# Autodesk Inventor assembly: Zlozenie_smc
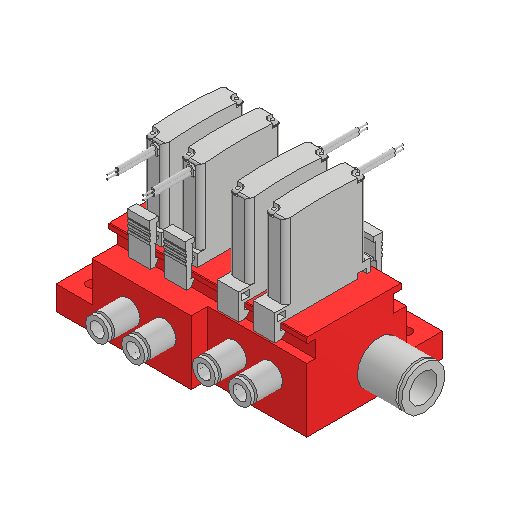
[picture p0: Inventor's stored thumbnail of the model, 512x512]
Saved by Autodesk Inventor 2024.3 (Build 283343000, 343)
## iProperties
Created: 2025-06-09
Part Number: Zlozenie_smc
Document SubType Name: Assembly
Designer: MPA
Author: MPA
## Documents named in this file (5)
- C:\MPA - shortPath\magisterka\V3\Workspace\Zlozenie_smc.iam
- C:\MPA - shortPath\magisterka\V3\Workspace\Zakupowe\smc\SX12F-KH.ipt
- C:\MPA - shortPath\magisterka\V3\Workspace\Plyta_SMC.ipt
- C:\MPA - shortPath\magisterka\V3\Workspace\Zakupowe\smc\KQ2S06-01AS_(A) Brass.ipt
- C:\MPA - shortPath\magisterka\V3\Workspace\Zakupowe\smc\KQ2S12-02AS_(A) Brass.ipt
## Components (10 placed, 4 different names)
1. Plyta_SMC:1 — Flush:1, Flush:2, Flush:3, Insert:1, Mate:1, Insert:2, Mate:2, Insert:3, Insert:4, Insert:5
2. KQ2S12-02AS_(A) Brass:1 — Insert:5
3. SX12F-KH:1 — Insert:1, Mate:1
4. SX12F-KH:2
5. SX12F-KH:3 — Insert:2, Mate:2
6. SX12F-KH:4
7. KQ2S06-01AS_(A) Brass:1 — Insert:3
8. KQ2S06-01AS_(A) Brass:2
9. KQ2S06-01AS_(A) Brass:3 — Insert:4
10. KQ2S06-01AS_(A) Brass:4
## Component patterns: (2 elements, first: SX12F-KH:1), (2 elements, first: SX12F-KH:3), (2 elements, first: KQ2S06-01AS_(A) Brass:1), (2 elements, first: KQ2S06-01AS_(A) Brass:3)
## Relationships (10: Insert 5, Flush 3, Mate 2)
- Flush:1: Plyta_SMC:1
- Flush:2: Plyta_SMC:1
- Flush:3: Plyta_SMC:1
- Insert:1: Plyta_SMC:1 ↔ SX12F-KH:1
- Mate:1: Plyta_SMC:1 ↔ SX12F-KH:1
- Insert:2: Plyta_SMC:1 ↔ SX12F-KH:3
- Mate:2: Plyta_SMC:1 ↔ SX12F-KH:3
- Insert:3: Plyta_SMC:1 ↔ KQ2S06-01AS_(A) Brass:1
- Insert:4: Plyta_SMC:1 ↔ KQ2S06-01AS_(A) Brass:3
- Insert:5: Plyta_SMC:1 ↔ KQ2S12-02AS_(A) Brass:1
